# Autodesk Inventor assembly: Robot
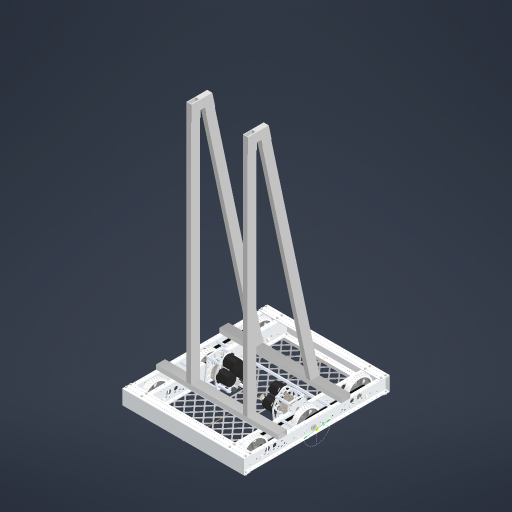
[picture p0: Inventor's stored thumbnail of the model, 512x512]
Saved by Autodesk Inventor 2023 (Build 270158000, 158)
## iProperties
Created: 2023-01-07
Part Number: Robot
Document SubType Name: Assembly
Designer: Blank Slate
Author: Blank Slate
## Documents named in this file (6)
- C:\Users\Terrence\Documents\FRC Long\Robot.iam
- C:\Users\Terrence\Documents\FRC Long\Parts\AM14U5 Long ToughBox Mini 6in HiGrip 6wD.iam
- C:\Users\Terrence\Documents\FRC Long\Parts\2+Stage+3+Motor+Evo+Shifter.iam
- C:\Users\Terrence\Documents\FRC Long\Parts\am-4258_15T NEO with 15T 32DP Pinion for EVO Gearboxes.ipt
- C:\Users\Terrence\Documents\FRC Long\Parts\bellypan.ipt
- C:\Users\Terrence\Documents\FRC Long\Truss.iam
## Components (11 placed, 5 different names)
1. AM14U5 Long ToughBox Mini 6in HiGrip 6wD:1 [sub-assembly] — Insert:13, Insert:14, Insert:15, Insert:16, Insert:17, Insert:18, Flush:1, Mate:1
2. 2+Stage+3+Motor+Evo+Shifter:1 [sub-assembly] — Insert:1, Insert:2, Insert:3, Insert:4, Insert:5, Insert:6, Insert:15, Insert:16
3. am-4258_15T NEO with 15T 32DP Pinion for EVO Gearboxes:1 — Insert:1, Insert:2
4. am-4258_15T NEO with 15T 32DP Pinion for EVO Gearboxes:2 — Insert:3, Insert:4
5. am-4258_15T NEO with 15T 32DP Pinion for EVO Gearboxes:3 — Insert:5, Insert:6
6. 2+Stage+3+Motor+Evo+Shifter:2 [sub-assembly] — Insert:13, Insert:14
7. am-4258_15T NEO with 15T 32DP Pinion for EVO Gearboxes:4
8. am-4258_15T NEO with 15T 32DP Pinion for EVO Gearboxes:5
9. am-4258_15T NEO with 15T 32DP Pinion for EVO Gearboxes:6
10. bellypan:1 — Insert:17, Insert:18
11. Truss:1 [sub-assembly] — Flush:1, Mate:1
## Relationships (20: Insert 18, Flush 1, Mate 1)
- Insert:1: 2+Stage+3+Motor+Evo+Shifter:1 ↔ am-4258_15T NEO with 15T 32DP Pinion for EVO Gearboxes:1
- Insert:2: 2+Stage+3+Motor+Evo+Shifter:1 ↔ am-4258_15T NEO with 15T 32DP Pinion for EVO Gearboxes:1
- Insert:3: 2+Stage+3+Motor+Evo+Shifter:1 ↔ am-4258_15T NEO with 15T 32DP Pinion for EVO Gearboxes:2
- Insert:4: 2+Stage+3+Motor+Evo+Shifter:1 ↔ am-4258_15T NEO with 15T 32DP Pinion for EVO Gearboxes:2
- Insert:5: 2+Stage+3+Motor+Evo+Shifter:1 ↔ am-4258_15T NEO with 15T 32DP Pinion for EVO Gearboxes:3
- Insert:6: 2+Stage+3+Motor+Evo+Shifter:1 ↔ am-4258_15T NEO with 15T 32DP Pinion for EVO Gearboxes:3
- [Insert]: 2+Stage+3+Motor+Evo+Shifter:2 ↔ am-4258_15T NEO with 15T 32DP Pinion for EVO Gearboxes:4
- [Insert]: 2+Stage+3+Motor+Evo+Shifter:2 ↔ am-4258_15T NEO with 15T 32DP Pinion for EVO Gearboxes:4
- [Insert]: 2+Stage+3+Motor+Evo+Shifter:2 ↔ am-4258_15T NEO with 15T 32DP Pinion for EVO Gearboxes:5
- [Insert]: 2+Stage+3+Motor+Evo+Shifter:2 ↔ am-4258_15T NEO with 15T 32DP Pinion for EVO Gearboxes:5
- [Insert]: 2+Stage+3+Motor+Evo+Shifter:2 ↔ am-4258_15T NEO with 15T 32DP Pinion for EVO Gearboxes:6
- [Insert]: 2+Stage+3+Motor+Evo+Shifter:2 ↔ am-4258_15T NEO with 15T 32DP Pinion for EVO Gearboxes:6
- Insert:13: AM14U5 Long ToughBox Mini 6in HiGrip 6wD:1 ↔ 2+Stage+3+Motor+Evo+Shifter:2
- Insert:14: AM14U5 Long ToughBox Mini 6in HiGrip 6wD:1 ↔ 2+Stage+3+Motor+Evo+Shifter:2
- Insert:15: AM14U5 Long ToughBox Mini 6in HiGrip 6wD:1 ↔ 2+Stage+3+Motor+Evo+Shifter:1
- Insert:16: AM14U5 Long ToughBox Mini 6in HiGrip 6wD:1 ↔ 2+Stage+3+Motor+Evo+Shifter:1
- Insert:17: AM14U5 Long ToughBox Mini 6in HiGrip 6wD:1 ↔ bellypan:1
- Insert:18: AM14U5 Long ToughBox Mini 6in HiGrip 6wD:1 ↔ bellypan:1
- Flush:1: AM14U5 Long ToughBox Mini 6in HiGrip 6wD:1 ↔ Truss:1
- Mate:1: AM14U5 Long ToughBox Mini 6in HiGrip 6wD:1 ↔ Truss:1
## Named parameters: d6_d0 = 0 mm, d7_d1 = 0 mm, d8_d2 = 0 mm, d9_d3 = 0 mm, d10_d4 = 0 mm, d11_d5 = 0 mm
